# Autodesk Inventor assembly: Chassis Assembly 26x28 Version
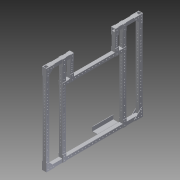
[picture p0: Inventor's stored thumbnail of the model, 180x180]
Saved by Autodesk Inventor 2013 (Build 170138000, 138)
## iProperties
Created: 2013-01-06
Part Number: Chassis Assembly 26x28 Version
Document SubType Name: Assembly
Designer: Moses
Mass: 3363.47 g
Surface Area: 8280.6 cm^2
Volume: 1241.13 cm^3
Density: 2.71 g/cm^3
Author: Moses
## Documents named in this file (11)
- C:\Users\Moses\Documents\GitHub\frc2013CAD\Chassis\Chassis Assembly 26x28 Version\Chassis Assembly 26x28 Version.iam
- C:\Users\Moses\Documents\GitHub\frc2013CAD\Chassis\Chassis V1.500 Part3-mirror.ipt
- C:\Users\Moses\Documents\GitHub\frc2013CAD\Chassis\Chassis V1.500 Part8.ipt
- C:\Users\Moses\Documents\GitHub\frc2013CAD\Chassis\Chassis V1.500 Part7.ipt
- C:\Users\Moses\Documents\GitHub\frc2013CAD\Chassis\Chassis V1.500 Part2.ipt
- C:\Users\Moses\Documents\GitHub\frc2013CAD\Chassis\Chassis V1.500 Part3.ipt
- C:\Users\Moses\Documents\GitHub\frc2013CAD\Chassis\Chassis Connector Plate V1.500.ipt
- C:\Users\Moses\Documents\GitHub\frc2013CAD\Chassis\Chassis Corner Plate V1.500.ipt
- C:\Users\Moses\Documents\GitHub\frc2013CAD\Chassis\Chassis Assembly 26x28 Version\Chassis Part4 (26x28).ipt
- C:\Users\Moses\Documents\GitHub\frc2013CAD\Chassis\Chassis Assembly 26x28 Version\Chassis Part1 (26x28).ipt
- C:\Users\Moses\Documents\GitHub\frc2013CAD\Chassis\Chassis Assembly 26x28 Version\Chassis Battery Mount Part1.ipt
## Components (39 placed, 10 different names)
1. Chassis Part1 (26x28):1 — Mate:2, Flush:3, Flush:4, Flush:12, Mate:6, Flush:21, Flush:22, Mate:14, Flush:23, Flush:24, Mate:15, Flush:26, Mate:16, Flush:27, Flush:28, Flush:25
2. Chassis Part1 (26x28):2 — Mate:3, Flush:5, Flush:6, Flush:10, Mate:5, Flush:17, Mate:17, Flush:29, Flush:30, Mate:18, Flush:31, Flush:32, Mate:19, Flush:33, Flush:34, Mate:20, Flush:35, Flush:36
3. Chassis V1.500 Part2:1 — Mate:2, Flush:3, Flush:4, Mate:3, Flush:5, Flush:6, Mate:8, Mate:9, Flush:15, Flush:16, Mate:24, Mate:25, Mate:27, Mate:28, Mate:36, Mate:37, Mate:39, Mate:40, Mate:76, Mate:77, Mate:78
4. Chassis Part4 (26x28):1 — Flush:10, Mate:4, Flush:13, Mate:8, Flush:16, Mate:23, Mate:26, Mate:35, Mate:38, Mate:45, Flush:37
5. Chassis Part4 (26x28):2 — Flush:12, Flush:14, Mate:7, Mate:9, Flush:15, Mate:29, Mate:32, Mate:41, Mate:44
6. Chassis V1.500 Part3-mirror:1 — Mate:4, Mate:5, Flush:13, Mate:21, Mate:22, Mate:33, Mate:34, Flush:38, Mate:54, Flush:43, Flush:44, Mate:58, Mate:61
7. Chassis V1.500 Part3:1 — Mate:6, Flush:14, Mate:7, Mate:13, Mate:30, Mate:31, Mate:42, Mate:43, Mate:55, Flush:45, Flush:46, Mate:64, Mate:67
8. Chassis Corner Plate V1.500:1 — Flush:21, Mate:13, Flush:22
9. Chassis Corner Plate V1.500:2 — Mate:14, Flush:23, Flush:24
10. Chassis Corner Plate V1.500:3 — Mate:15, Flush:25, Flush:26
11. Chassis Corner Plate V1.500:4 — Mate:16, Flush:27, Flush:28
12. Chassis Corner Plate V1.500:5 — Mate:17, Flush:29, Flush:30
13. Chassis Corner Plate V1.500:6 — Mate:18, Flush:31, Flush:32
14. Chassis Corner Plate V1.500:7 — Mate:19, Flush:33, Flush:34
15. Chassis Corner Plate V1.500:8 — Mate:20, Flush:35, Flush:36
16. Chassis Connector Plate V1.500:1 — Mate:21, Mate:22, Mate:23
17. Chassis Connector Plate V1.500:2 — Mate:24, Mate:25, Mate:26
18. Chassis Connector Plate V1.500:3 — Mate:27, Mate:28, Mate:29
19. Chassis Connector Plate V1.500:4 — Mate:30, Mate:31, Mate:32
20. Chassis Connector Plate V1.500:5 — Mate:33, Mate:34, Mate:35
21. Chassis Connector Plate V1.500:6 — Mate:36, Mate:37, Mate:38
22. Chassis Connector Plate V1.500:7 — Mate:39, Mate:40, Mate:41
23. Chassis Connector Plate V1.500:8 — Mate:42, Mate:43, Mate:44
24. Chassis V1.500 Part7:1 — Mate:45, Flush:37, Flush:38, Mate:46, Mate:47, Flush:39, Mate:48, Mate:49, Flush:40, Mate:50, Mate:51, Flush:41, Mate:52, Mate:53, Flush:42
25. Chassis Connector Plate V1.500:9 — Mate:52, Mate:53, Flush:42
26. Chassis Connector Plate V1.500:10 — Mate:50, Mate:51, Flush:41
27. Chassis Connector Plate V1.500:11 — Mate:48, Mate:49, Flush:40
28. Chassis Connector Plate V1.500:12 — Mate:46, Mate:47, Flush:39
29. Chassis V1.500 Part8:1 — Mate:54, Flush:43, Flush:44, Mate:56, Mate:57, Mate:59, Mate:60, Mate:68, Mate:69, Flush:47, Mate:70, Mate:71, Flush:48
30. Chassis V1.500 Part8:2 — Mate:55, Flush:45, Flush:46, Mate:62, Mate:63, Mate:65, Mate:66, Mate:72, Mate:73, Mate:74, Mate:75, Flush:49, Flush:50
31. Chassis Connector Plate V1.500:13 — Mate:56, Mate:57, Mate:58
32. Chassis Connector Plate V1.500:14 — Mate:59, Mate:60, Mate:61
33. Chassis Connector Plate V1.500:15 — Mate:65, Mate:66, Mate:67
34. Chassis Connector Plate V1.500:16 — Mate:62, Mate:63, Mate:64
35. Chassis Connector Plate V1.500:17 — Mate:68, Mate:69, Flush:47
36. Chassis Connector Plate V1.500:18 — Mate:70, Mate:71, Flush:48
37. Chassis Connector Plate V1.500:19 — Mate:72, Mate:73, Flush:50
38. Chassis Connector Plate V1.500:20 — Mate:74, Mate:75, Flush:49
39. Chassis Battery Mount Part1:1 — Mate:76, Mate:77, Mate:78
## Relationships (115: Mate 74, Flush 41)
- Mate:2: Chassis Part1 (26x28):1 ↔ Chassis V1.500 Part2:1
- Flush:3: Chassis Part1 (26x28):1 ↔ Chassis V1.500 Part2:1
- Flush:4: Chassis Part1 (26x28):1 ↔ Chassis V1.500 Part2:1
- Mate:3: Chassis Part1 (26x28):2 ↔ Chassis V1.500 Part2:1
- Flush:5: Chassis Part1 (26x28):2 ↔ Chassis V1.500 Part2:1
- Flush:6: Chassis Part1 (26x28):2 ↔ Chassis V1.500 Part2:1
- Flush:10 (-120.65 mm): Chassis Part1 (26x28):2 ↔ Chassis Part4 (26x28):1
- Flush:12 (-120.65 mm): Chassis Part1 (26x28):1 ↔ Chassis Part4 (26x28):2
- Mate:4: Chassis Part4 (26x28):1 ↔ Chassis V1.500 Part3-mirror:1
- Mate:5: Chassis Part1 (26x28):2 ↔ Chassis V1.500 Part3-mirror:1
- Flush:13: Chassis Part4 (26x28):1 ↔ Chassis V1.500 Part3-mirror:1
- Mate:6: Chassis Part1 (26x28):1 ↔ Chassis V1.500 Part3:1
- Flush:14: Chassis Part4 (26x28):2 ↔ Chassis V1.500 Part3:1
- Mate:7: Chassis Part4 (26x28):2 ↔ Chassis V1.500 Part3:1
- Mate:8: Chassis V1.500 Part2:1 ↔ Chassis Part4 (26x28):1
- Mate:9: Chassis V1.500 Part2:1 ↔ Chassis Part4 (26x28):2
- Flush:15: Chassis V1.500 Part2:1 ↔ Chassis Part4 (26x28):2
- Flush:16: Chassis V1.500 Part2:1 ↔ Chassis Part4 (26x28):1
- Flush:17 (330.2 mm): Chassis Part1 (26x28):2
- Flush:21: Chassis Part1 (26x28):1 ↔ Chassis Corner Plate V1.500:1
- Mate:13: Chassis V1.500 Part3:1 ↔ Chassis Corner Plate V1.500:1
- Flush:22: Chassis Part1 (26x28):1 ↔ Chassis Corner Plate V1.500:1
- Mate:14: Chassis Part1 (26x28):1 ↔ Chassis Corner Plate V1.500:2
- Flush:23: Chassis Part1 (26x28):1 ↔ Chassis Corner Plate V1.500:2
- Flush:24: Chassis Part1 (26x28):1 ↔ Chassis Corner Plate V1.500:2
- Mate:15: Chassis Part1 (26x28):1 ↔ Chassis Corner Plate V1.500:3
- Flush:25: Chassis Part1 (26x28):1 ↔ Chassis Corner Plate V1.500:3
- Flush:26: Chassis Part1 (26x28):1 ↔ Chassis Corner Plate V1.500:3
- Mate:16: Chassis Part1 (26x28):1 ↔ Chassis Corner Plate V1.500:4
- Flush:27: Chassis Part1 (26x28):1 ↔ Chassis Corner Plate V1.500:4
- Flush:28: Chassis Part1 (26x28):1 ↔ Chassis Corner Plate V1.500:4
- Mate:17: Chassis Part1 (26x28):2 ↔ Chassis Corner Plate V1.500:5
- Flush:29: Chassis Part1 (26x28):2 ↔ Chassis Corner Plate V1.500:5
- Flush:30: Chassis Part1 (26x28):2 ↔ Chassis Corner Plate V1.500:5
- Mate:18: Chassis Part1 (26x28):2 ↔ Chassis Corner Plate V1.500:6
- Flush:31: Chassis Part1 (26x28):2 ↔ Chassis Corner Plate V1.500:6
- Flush:32: Chassis Part1 (26x28):2 ↔ Chassis Corner Plate V1.500:6
- Mate:19: Chassis Part1 (26x28):2 ↔ Chassis Corner Plate V1.500:7
- Flush:33: Chassis Part1 (26x28):2 ↔ Chassis Corner Plate V1.500:7
- Flush:34: Chassis Part1 (26x28):2 ↔ Chassis Corner Plate V1.500:7
- Mate:20: Chassis Part1 (26x28):2 ↔ Chassis Corner Plate V1.500:8
- Flush:35: Chassis Part1 (26x28):2 ↔ Chassis Corner Plate V1.500:8
- Flush:36: Chassis Part1 (26x28):2 ↔ Chassis Corner Plate V1.500:8
- Mate:21: Chassis V1.500 Part3-mirror:1 ↔ Chassis Connector Plate V1.500:1
- Mate:22: Chassis V1.500 Part3-mirror:1 ↔ Chassis Connector Plate V1.500:1
- Mate:23: Chassis Part4 (26x28):1 ↔ Chassis Connector Plate V1.500:1
- Mate:24: Chassis V1.500 Part2:1 ↔ Chassis Connector Plate V1.500:2
- Mate:25: Chassis V1.500 Part2:1 ↔ Chassis Connector Plate V1.500:2
- Mate:26: Chassis Part4 (26x28):1 ↔ Chassis Connector Plate V1.500:2
- Mate:27: Chassis V1.500 Part2:1 ↔ Chassis Connector Plate V1.500:3
- Mate:28: Chassis V1.500 Part2:1 ↔ Chassis Connector Plate V1.500:3
- Mate:29: Chassis Part4 (26x28):2 ↔ Chassis Connector Plate V1.500:3
- Mate:30: Chassis V1.500 Part3:1 ↔ Chassis Connector Plate V1.500:4
- Mate:31: Chassis V1.500 Part3:1 ↔ Chassis Connector Plate V1.500:4
- Mate:32: Chassis Part4 (26x28):2 ↔ Chassis Connector Plate V1.500:4
- Mate:33: Chassis V1.500 Part3-mirror:1 ↔ Chassis Connector Plate V1.500:5
- Mate:34: Chassis V1.500 Part3-mirror:1 ↔ Chassis Connector Plate V1.500:5
- Mate:35: Chassis Part4 (26x28):1 ↔ Chassis Connector Plate V1.500:5
- Mate:36: Chassis V1.500 Part2:1 ↔ Chassis Connector Plate V1.500:6
- Mate:37: Chassis V1.500 Part2:1 ↔ Chassis Connector Plate V1.500:6
- Mate:38: Chassis Part4 (26x28):1 ↔ Chassis Connector Plate V1.500:6
- Mate:39: Chassis V1.500 Part2:1 ↔ Chassis Connector Plate V1.500:7
- Mate:40: Chassis V1.500 Part2:1 ↔ Chassis Connector Plate V1.500:7
- Mate:41: Chassis Part4 (26x28):2 ↔ Chassis Connector Plate V1.500:7
- Mate:42: Chassis V1.500 Part3:1 ↔ Chassis Connector Plate V1.500:8
- Mate:43: Chassis V1.500 Part3:1 ↔ Chassis Connector Plate V1.500:8
- Mate:44: Chassis Part4 (26x28):2 ↔ Chassis Connector Plate V1.500:8
- Mate:45: Chassis Part4 (26x28):1 ↔ Chassis V1.500 Part7:1
- Flush:37: Chassis Part4 (26x28):1 ↔ Chassis V1.500 Part7:1
- Flush:38 (-152.4 mm): Chassis V1.500 Part3-mirror:1 ↔ Chassis V1.500 Part7:1
- Mate:46: Chassis V1.500 Part7:1 ↔ Chassis Connector Plate V1.500:12
- Mate:47: Chassis V1.500 Part7:1 ↔ Chassis Connector Plate V1.500:12
- Flush:39: Chassis V1.500 Part7:1 ↔ Chassis Connector Plate V1.500:12
- Mate:48: Chassis V1.500 Part7:1 ↔ Chassis Connector Plate V1.500:11
- Mate:49: Chassis V1.500 Part7:1 ↔ Chassis Connector Plate V1.500:11
- Flush:40: Chassis V1.500 Part7:1 ↔ Chassis Connector Plate V1.500:11
- Mate:50: Chassis V1.500 Part7:1 ↔ Chassis Connector Plate V1.500:10
- Mate:51: Chassis V1.500 Part7:1 ↔ Chassis Connector Plate V1.500:10
- Flush:41: Chassis V1.500 Part7:1 ↔ Chassis Connector Plate V1.500:10
- Mate:52: Chassis V1.500 Part7:1 ↔ Chassis Connector Plate V1.500:9
- Mate:53: Chassis V1.500 Part7:1 ↔ Chassis Connector Plate V1.500:9
- Flush:42: Chassis V1.500 Part7:1 ↔ Chassis Connector Plate V1.500:9
- Mate:54: Chassis V1.500 Part3-mirror:1 ↔ Chassis V1.500 Part8:1
- Flush:43: Chassis V1.500 Part3-mirror:1 ↔ Chassis V1.500 Part8:1
- Flush:44: Chassis V1.500 Part3-mirror:1 ↔ Chassis V1.500 Part8:1
- Mate:55: Chassis V1.500 Part3:1 ↔ Chassis V1.500 Part8:2
- Flush:45: Chassis V1.500 Part3:1 ↔ Chassis V1.500 Part8:2
- Flush:46: Chassis V1.500 Part3:1 ↔ Chassis V1.500 Part8:2
- Mate:56: Chassis V1.500 Part8:1 ↔ Chassis Connector Plate V1.500:13
- Mate:57: Chassis V1.500 Part8:1 ↔ Chassis Connector Plate V1.500:13
- Mate:58: Chassis V1.500 Part3-mirror:1 ↔ Chassis Connector Plate V1.500:13
- Mate:59: Chassis V1.500 Part8:1 ↔ Chassis Connector Plate V1.500:14
- Mate:60: Chassis V1.500 Part8:1 ↔ Chassis Connector Plate V1.500:14
- Mate:61: Chassis V1.500 Part3-mirror:1 ↔ Chassis Connector Plate V1.500:14
- Mate:62: Chassis V1.500 Part8:2 ↔ Chassis Connector Plate V1.500:16
- Mate:63: Chassis V1.500 Part8:2 ↔ Chassis Connector Plate V1.500:16
- Mate:64: Chassis V1.500 Part3:1 ↔ Chassis Connector Plate V1.500:16
- Mate:65: Chassis V1.500 Part8:2 ↔ Chassis Connector Plate V1.500:15
- Mate:66: Chassis V1.500 Part8:2 ↔ Chassis Connector Plate V1.500:15
- Mate:67: Chassis V1.500 Part3:1 ↔ Chassis Connector Plate V1.500:15
- Mate:68: Chassis V1.500 Part8:1 ↔ Chassis Connector Plate V1.500:17
- Mate:69: Chassis V1.500 Part8:1 ↔ Chassis Connector Plate V1.500:17
- Flush:47: Chassis V1.500 Part8:1 ↔ Chassis Connector Plate V1.500:17
- Mate:70: Chassis V1.500 Part8:1 ↔ Chassis Connector Plate V1.500:18
- Mate:71: Chassis V1.500 Part8:1 ↔ Chassis Connector Plate V1.500:18
- Flush:48: Chassis V1.500 Part8:1 ↔ Chassis Connector Plate V1.500:18
- Mate:72: Chassis V1.500 Part8:2 ↔ Chassis Connector Plate V1.500:19
- Mate:73: Chassis V1.500 Part8:2 ↔ Chassis Connector Plate V1.500:19
- Mate:74: Chassis V1.500 Part8:2 ↔ Chassis Connector Plate V1.500:20
- Mate:75: Chassis V1.500 Part8:2 ↔ Chassis Connector Plate V1.500:20
- Flush:49: Chassis V1.500 Part8:2 ↔ Chassis Connector Plate V1.500:20
- Flush:50: Chassis V1.500 Part8:2 ↔ Chassis Connector Plate V1.500:19
- Mate:76: Chassis V1.500 Part2:1 ↔ Chassis Battery Mount Part1:1
- Mate:77: Chassis V1.500 Part2:1 ↔ Chassis Battery Mount Part1:1
- Mate:78: Chassis V1.500 Part2:1 ↔ Chassis Battery Mount Part1:1
